# Autodesk Inventor assembly: shoulder_link
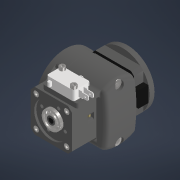
[picture p0: Inventor's stored thumbnail of the model, 180x180]
Saved by Autodesk Inventor 2022 (Build 260153070, 153G)
## iProperties
Created: 2021-11-21
Part Number: shoulder_link
Document SubType Name: Assembly
Designer: Teo
Title: Predstavitev sklopa
Author: Teo
## Documents named in this file (13)
- D:\Zaključna\Roka\Priloge\IPT_files\Assemblies\shoulder_link.iam
- D:\Zaključna\Roka\Priloge\IPT_files\Stepper_nema17.ipt
- D:\Zaključna\Roka\Priloge\IPT_files\Rotor_lite.ipt
- C:\Users\Teo\Documents\Inventor\Content Center Files\R2022\en-US\DIN 912\DIN 912 - M4 x 0.7 x 12 x 10.25.ipt
- D:\Zaključna\Roka\Priloge\IPT_files\Assemblies\reductor.iam
- D:\Zaključna\Roka\Priloge\IPT_files\Bearing_back_lite.ipt
- C:\Users\Teo\Documents\Inventor\Content Center Files\R2022\en-US\DIN 912\DIN 912 - M3 x 0.5 x 30 x 18.ipt
- C:\Users\Teo\Documents\Inventor\Content Center Files\R2022\en-US\DIN 912\DIN 912 - M3 x 0.5 x 25 x 18.ipt
- C:\Users\Teo\Documents\Inventor\Content Center Files\R2022\en-US\DIN 625 - T1\DIN 625 T1 - 619_8 - 8 x 19 x 6.ipt
- D:\Zaključna\Roka\Priloge\IPT_files\Stepper_bracket_1_lite.ipt
- C:\Users\Teo\Documents\Inventor\Content Center Files\R2022\en-US\DIN 912\DIN 912 - M5 x 0.8 x 40 x 22.ipt
- D:\Zaključna\Roka\Priloge\IPT_files\Limit_switch.ipt
- C:\Users\Teo\Documents\Inventor\Content Center Files\R2022\en-US\DIN 912\DIN 912 - M3 x 0.5 x 12 x 10.75.ipt
## Components (23 placed, 12 different names)
1. Stepper_nema17:1 — Mate:11, Mate:12, Mate:13, Mate:14, Mate:15, Mate:18, Mate:20, Mate:22, Mate:24, Mate:37, Mate:38, Mate:41
2. Rotor_lite:1 — Mate:1, Mate:2, Mate:3, Mate:4, Mate:5, Mate:6, Mate:7, Mate:8, Mate:36, Mate:37, Mate:38, Mate:42, Mate:43, Mate:44, Mate:46
3. reductor:1 [sub-assembly] — Mate:11, Mate:12, Mate:13, Mate:14, Mate:26, Mate:27, Mate:28, Mate:29, Mate:30, Mate:31, Mate:32, Mate:33, Symmetry:1
4. Bearing_back_lite:1 — Mate:15, Mate:19, Mate:21, Mate:23, Mate:25, Mate:34, Mate:35, Mate:39, Mate:40
5. Stepper_bracket_1_lite:1 — Mate:41, Mate:42, Mate:43, Mate:45, Mate:47, Mate:48, Mate:49, Angle:1, Mate:50, Mate:52
6. Limit_switch:1 — Mate:48, Mate:49, Angle:1, Mate:51, Mate:53
7. DIN 912 - replaced by DIN EN ISO 4762 M3 x 12:1 — Mate:50, Mate:51
8. DIN 912 - replaced by DIN EN ISO 4762 M3 x 12:2 — Mate:52, Mate:53
9. DIN 912 - replaced by DIN EN ISO 4762 M5 x 40:2 — Mate:46, Mate:47
10. DIN 912 - replaced by DIN EN ISO 4762 M5 x 40:1 — Mate:44, Mate:45
11. DIN 912 - replaced by DIN EN ISO 4762 M3 x 25:3 — Mate:32, Mate:33
12. DIN 625 - T1 619/8 - 8 x 19 x 6:1 — Mate:34, Mate:35, Symmetry:1
13. DIN 912 - replaced by DIN EN ISO 4762 M3 x 25:2 — Mate:30, Mate:31
14. DIN 912 - replaced by DIN EN ISO 4762 M3 x 25:1 — Mate:28, Mate:29
15. DIN 912 - replaced by DIN EN ISO 4762 M3 x 25:4 — Mate:26, Mate:27
16. DIN 912 - replaced by DIN EN ISO 4762 M3 x 30:2 — Mate:24, Mate:25, Mate:40
17. DIN 912 - replaced by DIN EN ISO 4762 M3 x 30:4 — Mate:22, Mate:23, Mate:39
18. DIN 912 - replaced by DIN EN ISO 4762 M3 x 30:3 — Mate:20, Mate:21
19. DIN 912 - replaced by DIN EN ISO 4762 M3 x 30:1 — Mate:18, Mate:19
20. DIN 912 - replaced by DIN EN ISO 4762 M4 x 12:3 — Mate:7, Mate:8
21. DIN 912 - replaced by DIN EN ISO 4762 M4 x 12:4 — Mate:5, Mate:6
22. DIN 912 - replaced by DIN EN ISO 4762 M4 x 12:2 — Mate:3, Mate:4
23. DIN 912 - replaced by DIN EN ISO 4762 M4 x 12:1 — Mate:1, Mate:2
## Relationships (51: Mate 49, Symmetry 1, Angle 1)
- Mate:1: Rotor_lite:1 ↔ DIN 912 - replaced by DIN EN ISO 4762 M4 x 12:1
- Mate:2: Rotor_lite:1 ↔ DIN 912 - replaced by DIN EN ISO 4762 M4 x 12:1
- Mate:3: Rotor_lite:1 ↔ DIN 912 - replaced by DIN EN ISO 4762 M4 x 12:2
- Mate:4: Rotor_lite:1 ↔ DIN 912 - replaced by DIN EN ISO 4762 M4 x 12:2
- Mate:5: Rotor_lite:1 ↔ DIN 912 - replaced by DIN EN ISO 4762 M4 x 12:4
- Mate:6: Rotor_lite:1 ↔ DIN 912 - replaced by DIN EN ISO 4762 M4 x 12:4
- Mate:7: Rotor_lite:1 ↔ DIN 912 - replaced by DIN EN ISO 4762 M4 x 12:3
- Mate:8: Rotor_lite:1 ↔ DIN 912 - replaced by DIN EN ISO 4762 M4 x 12:3
- Mate:11: Stepper_nema17:1 ↔ reductor:1
- Mate:12: Stepper_nema17:1 ↔ reductor:1
- Mate:13: Stepper_nema17:1 ↔ reductor:1
- Mate:14: Stepper_nema17:1 ↔ reductor:1
- Mate:15: Stepper_nema17:1 ↔ Bearing_back_lite:1
- Mate:18: Stepper_nema17:1 ↔ DIN 912 - replaced by DIN EN ISO 4762 M3 x 30:1
- Mate:19: Bearing_back_lite:1 ↔ DIN 912 - replaced by DIN EN ISO 4762 M3 x 30:1
- Mate:20: Stepper_nema17:1 ↔ DIN 912 - replaced by DIN EN ISO 4762 M3 x 30:3
- Mate:21: Bearing_back_lite:1 ↔ DIN 912 - replaced by DIN EN ISO 4762 M3 x 30:3
- Mate:22: Stepper_nema17:1 ↔ DIN 912 - replaced by DIN EN ISO 4762 M3 x 30:4
- Mate:23: Bearing_back_lite:1 ↔ DIN 912 - replaced by DIN EN ISO 4762 M3 x 30:4
- Mate:24: Stepper_nema17:1 ↔ DIN 912 - replaced by DIN EN ISO 4762 M3 x 30:2
- Mate:25: Bearing_back_lite:1 ↔ DIN 912 - replaced by DIN EN ISO 4762 M3 x 30:2
- Mate:26: reductor:1 ↔ DIN 912 - replaced by DIN EN ISO 4762 M3 x 25:4
- Mate:27: reductor:1 ↔ DIN 912 - replaced by DIN EN ISO 4762 M3 x 25:4
- Mate:28: reductor:1 ↔ DIN 912 - replaced by DIN EN ISO 4762 M3 x 25:1
- Mate:29: reductor:1 ↔ DIN 912 - replaced by DIN EN ISO 4762 M3 x 25:1
- Mate:30: reductor:1 ↔ DIN 912 - replaced by DIN EN ISO 4762 M3 x 25:2
- Mate:31: reductor:1 ↔ DIN 912 - replaced by DIN EN ISO 4762 M3 x 25:2
- Mate:32: reductor:1 ↔ DIN 912 - replaced by DIN EN ISO 4762 M3 x 25:3
- Mate:33: reductor:1 ↔ DIN 912 - replaced by DIN EN ISO 4762 M3 x 25:3
- Mate:34: Bearing_back_lite:1 ↔ DIN 625 - T1 619/8 - 8 x 19 x 6:1
- Mate:35: Bearing_back_lite:1 ↔ DIN 625 - T1 619/8 - 8 x 19 x 6:1
- Symmetry:1: reductor:1 ↔ DIN 625 - T1 619/8 - 8 x 19 x 6:1
- Mate:36: Rotor_lite:1
- Mate:37: Stepper_nema17:1 ↔ Rotor_lite:1
- Mate:38: Stepper_nema17:1 ↔ Rotor_lite:1
- Mate:39: Bearing_back_lite:1 ↔ DIN 912 - replaced by DIN EN ISO 4762 M3 x 30:4
- Mate:40: Bearing_back_lite:1 ↔ DIN 912 - replaced by DIN EN ISO 4762 M3 x 30:2
- Mate:41: Stepper_nema17:1 ↔ Stepper_bracket_1_lite:1
- Mate:42: Rotor_lite:1 ↔ Stepper_bracket_1_lite:1
- Mate:43: Rotor_lite:1 ↔ Stepper_bracket_1_lite:1
- Mate:44: Rotor_lite:1 ↔ DIN 912 - replaced by DIN EN ISO 4762 M5 x 40:1
- Mate:45: Stepper_bracket_1_lite:1 ↔ DIN 912 - replaced by DIN EN ISO 4762 M5 x 40:1
- Mate:46: Rotor_lite:1 ↔ DIN 912 - replaced by DIN EN ISO 4762 M5 x 40:2
- Mate:47: Stepper_bracket_1_lite:1 ↔ DIN 912 - replaced by DIN EN ISO 4762 M5 x 40:2
- Mate:48: Stepper_bracket_1_lite:1 ↔ Limit_switch:1
- Mate:49: Stepper_bracket_1_lite:1 ↔ Limit_switch:1
- Angle:1 (0 deg): Stepper_bracket_1_lite:1 ↔ Limit_switch:1
- Mate:50: Stepper_bracket_1_lite:1 ↔ DIN 912 - replaced by DIN EN ISO 4762 M3 x 12:1
- Mate:51: Limit_switch:1 ↔ DIN 912 - replaced by DIN EN ISO 4762 M3 x 12:1
- Mate:52: Stepper_bracket_1_lite:1 ↔ DIN 912 - replaced by DIN EN ISO 4762 M3 x 12:2
- Mate:53: Limit_switch:1 ↔ DIN 912 - replaced by DIN EN ISO 4762 M3 x 12:2
